# Autodesk Inventor assembly: Full_Design
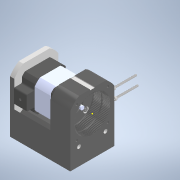
[picture p0: Inventor's stored thumbnail of the model, 180x180]
Saved by Autodesk Inventor 2022 (Build 260153000, 153)
## iProperties
Created: 2022-02-10
Part Number: Full_Design
Document SubType Name: Assembly
Designer: Mlees
Author: Mlees
## Documents named in this file (7)
- C:\Users\Mlees\Desktop\504Engineering\Stepper-Servo_Based_Robotic_Arm\Designs\Version_7\Full_Design.iam
- C:\Users\Mlees\Desktop\504Engineering\Stepper-Servo_Based_Robotic_Arm\Designs\Version_7\Downloaded_Parts\124125202-9-stp-mtr-17040w\stp-mtr-17040w.ipt
- C:\Users\Mlees\Desktop\504Engineering\Stepper-Servo_Based_Robotic_Arm\Designs\Version_7\Created_Parts\Combined_Gear_Box.ipt
- C:\Users\Mlees\Desktop\504Engineering\Stepper-Servo_Based_Robotic_Arm\Designs\Version_7\Created_Parts\Combined_Gear_Box_Modified.ipt
- C:\Users\Mlees\Desktop\504Engineering\Stepper-Servo_Based_Robotic_Arm\Designs\Version_7\Downloaded_Parts\nema17-speed-reducer-1.snapshot.9\M3 Insert 5D x 6L.step.ipt
- C:\Users\Mlees\Desktop\504Engineering\Stepper-Servo_Based_Robotic_Arm\Designs\Version_7\Downloaded_Parts\91290A101_Black-Oxide Alloy Steel Socket Head Screw_M3_6mm.ipt
- C:\Users\Mlees\Desktop\504Engineering\Stepper-Servo_Based_Robotic_Arm\Designs\Version_7\Downloaded_Parts\91290A059_Black-Oxide Alloy Steel Socket Head Screw_M3_30mm.ipt
## Components (15 placed, 6 different names)
1. Combined_Gear_Box:1 — Rigid:1, Rigid:2, Rigid:3, Rigid:4, Rigid:7, Rigid:8, Rotational:1, Rotational:2, Rotational:3, Rotational:4
2. Combined_Gear_Box_Modified:1 — Rigid:5, Rigid:6, Rigid:7
3. M3 Insert 5D x 6L.step:1 — Rigid:2
4. M3 Insert 5D x 6L.step:2 — Rigid:1
5. M3 Insert 5D x 6L.step:3 — Rigid:3
6. M3 Insert 5D x 6L.step:4 — Rigid:4
7. M3 Insert 5D x 6L.step:5 — Rigid:6
8. M3 Insert 5D x 6L.step:6 — Rigid:5
9. stp-mtr-17040w:1 — Rigid:8
10. 91290A101_Black-Oxide Alloy Steel Socket Head Screw_M3_6mm:1 — Rotational:1
11. 91290A101_Black-Oxide Alloy Steel Socket Head Screw_M3_6mm:2 — Rotational:2
12. 91290A101_Black-Oxide Alloy Steel Socket Head Screw_M3_6mm:3 — Rotational:3
13. 91290A101_Black-Oxide Alloy Steel Socket Head Screw_M3_6mm:4 — Rotational:4
14. 91290A059_Black-Oxide Alloy Steel Socket Head Screw_M3_30mm:1
15. 91290A059_Black-Oxide Alloy Steel Socket Head Screw_M3_30mm:2
## Relationships (12: WeldJoint 8, RevoluteJoint 4)
- Rigid:1 [WeldJoint]: Combined_Gear_Box:1 ↔ M3 Insert 5D x 6L.step:2
- Rigid:2 [WeldJoint]: Combined_Gear_Box:1 ↔ M3 Insert 5D x 6L.step:1
- Rigid:3 [WeldJoint]: Combined_Gear_Box:1 ↔ M3 Insert 5D x 6L.step:3
- Rigid:4 [WeldJoint]: Combined_Gear_Box:1 ↔ M3 Insert 5D x 6L.step:4
- Rigid:5 [WeldJoint]: Combined_Gear_Box_Modified:1 ↔ M3 Insert 5D x 6L.step:6
- Rigid:6 [WeldJoint]: Combined_Gear_Box_Modified:1 ↔ M3 Insert 5D x 6L.step:5
- Rigid:7 [WeldJoint]: Combined_Gear_Box:1 ↔ Combined_Gear_Box_Modified:1
- Rigid:8 [WeldJoint]: Combined_Gear_Box:1 ↔ stp-mtr-17040w:1
- Rotational:1 [RevoluteJoint]: Combined_Gear_Box:1 ↔ 91290A101_Black-Oxide Alloy Steel Socket Head Screw_M3_6mm:1
- Rotational:2 [RevoluteJoint]: Combined_Gear_Box:1 ↔ 91290A101_Black-Oxide Alloy Steel Socket Head Screw_M3_6mm:2
- Rotational:3 [RevoluteJoint]: Combined_Gear_Box:1 ↔ 91290A101_Black-Oxide Alloy Steel Socket Head Screw_M3_6mm:3
- Rotational:4 [RevoluteJoint]: Combined_Gear_Box:1 ↔ 91290A101_Black-Oxide Alloy Steel Socket Head Screw_M3_6mm:4
